# Autodesk Inventor assembly: Chassis
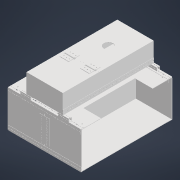
[picture p0: Inventor's stored thumbnail of the model, 180x180]
Saved by Autodesk Inventor 2022 (Build 260153000, 153)
## iProperties
Created: 2021-11-11
Part Number: Chassis
Document SubType Name: Assembly
Designer: 17185
Author: 17185
## Documents named in this file (4)
- G:\__projects\ROBOTICS\RCR\Chassis\Chassis Frame\Chassis.iam
- G:\__projects\ROBOTICS\RCR\Chassis\Chassis Frame\ChassisFrame.iam
- G:\__projects\ROBOTICS\RCR\Chassis\Chassis Frame\DriveHousing.iam
- G:\__projects\ROBOTICS\RCR\Chassis\Chassis Frame\ElectronicsHousing.iam
## Components (4 placed, 3 different names)
1. ChassisFrame:1 [sub-assembly] — Mate:1, Mate:2, Mate:3, Mate:4, Mate:5, Mate:6, Mate:7, Mate:8
2. DriveHousing:1 [sub-assembly] — Mate:1, Mate:2, Mate:3, Flush:1
3. DriveHousing:2 [sub-assembly] — Mate:4, Mate:5, Mate:6
4. ElectronicsHousing:1 [sub-assembly] — Mate:7, Flush:1, Mate:8
## Relationships (9: Mate 8, Flush 1)
- Mate:1: ChassisFrame:1 ↔ DriveHousing:1
- Mate:2: ChassisFrame:1 ↔ DriveHousing:1
- Mate:3: ChassisFrame:1 ↔ DriveHousing:1
- Mate:4: ChassisFrame:1 ↔ DriveHousing:2
- Mate:5: ChassisFrame:1 ↔ DriveHousing:2
- Mate:6: ChassisFrame:1 ↔ DriveHousing:2
- Mate:7: ChassisFrame:1 ↔ ElectronicsHousing:1
- Flush:1: DriveHousing:1 ↔ ElectronicsHousing:1
- Mate:8: ChassisFrame:1 ↔ ElectronicsHousing:1
